# Autodesk Inventor assembly: inner
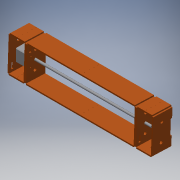
[picture p0: Inventor's stored thumbnail of the model, 180x180]
Saved by Autodesk Inventor 2017 (Build 210142000, 142)
## iProperties
Created: 2016-06-11
Part Number: inner
Document SubType Name: Assembly
Designer: daniel
Author: daniel
## Documents named in this file (7)
- C:\Users\daniel\Documents\GitHub\cardboard-stage-metric\stage\inner.iam
- C:\Users\daniel\Documents\GitHub\cardboard-stage-metric\stage\b1.iam
- C:\Users\daniel\Documents\GitHub\cardboard-stage-metric\stage\b3.iam
- C:\Users\daniel\Documents\GitHub\cardboard-stage-metric\stage\b5.iam
- C:\Users\daniel\Documents\GitHub\cardboard-stage-metric\stage\b2.iam
- C:\Users\daniel\Documents\GitHub\cardboard-stage-metric\stage\b4.iam
- C:\Users\daniel\Documents\GitHub\cardboard-stage-metric\stage\nema17_threaded_rod.ipt
## Components (7 placed, 6 different names)
1. b1:1 [sub-assembly] — Mate:5, Flush:9
2. nema17_threaded_rod:1 — Insert:1
3. b3:1 [sub-assembly] — Flush:10
4. b5:1 [sub-assembly] — Insert:1
5. b2:1 [sub-assembly] — Mate:3, Flush:5, Flush:6, Flush:7, Mate:5
6. b3:2 [sub-assembly] — Mate:3, Flush:5, Flush:6, Mate:4, Flush:8, Flush:9, Flush:10
7. b4:1 [sub-assembly] — Flush:7, Mate:4, Flush:8
## Relationships (16: Flush 10, Mate 5, Insert 1)
- [Flush]: b1:1 ↔ b5:1
- [Flush]: b1:1 ↔ b5:1
- [Mate]: b1:1 ↔ b5:1
- [Flush]: b3:1 ↔ b5:1
- [Mate]: b3:1 ↔ b5:1
- [Flush]: b3:1 ↔ b5:1
- Mate:3: b2:1 ↔ b3:2
- Flush:5: b2:1 ↔ b3:2
- Flush:6: b2:1 ↔ b3:2
- Flush:7: b2:1 ↔ b4:1
- Mate:4: b3:2 ↔ b4:1
- Flush:8: b3:2 ↔ b4:1
- Mate:5: b1:1 ↔ b2:1
- Flush:9: b1:1 ↔ b3:2
- Flush:10: b3:1 ↔ b3:2
- Insert:1: nema17_threaded_rod:1 ↔ b5:1
